# Autodesk Inventor assembly: joint4
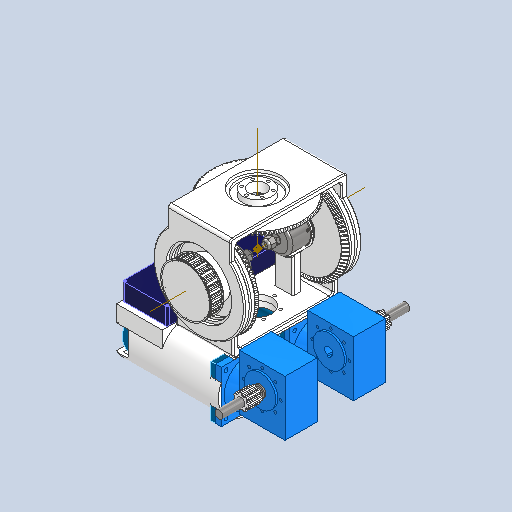
[picture p0: Inventor's stored thumbnail of the model, 512x512]
Saved by Autodesk Inventor 2025.3 (Build 293356030, 356C)
## iProperties
Created: 2025-08-31
Part Number: joint4
Document SubType Name: Assembly
Designer: MSI
Mass: 16772.4 g
Surface Area: 9850.81 cm^2
Volume: 6074.34 cm^3
Density: 2.76119 g/cm^3
Author: MSI
## Documents named in this file (14)
- C:\Users\MSI\Desktop\Project\11. 로봇팔\Robot Arm Model\Robot_Arm_6_v1\joint4.iam
- C:\Users\MSI\Desktop\Project\11. 로봇팔\Robot Arm Model\Robot_Arm_6_v1\motor_holder_1.ipt
- C:\Users\MSI\Desktop\Project\11. 로봇팔\Robot Arm Model\Robot_Arm_6_v1\NMRV30_motor.iam
- C:\Users\MSI\Desktop\Project\11. 로봇팔\Robot Arm Model\Robot_Arm_6_v1\base.ipt
- C:\Users\MSI\Desktop\Project\11. 로봇팔\Robot Arm Model\Robot_Arm_6_v1\frame.ipt
- C:\Users\MSI\Desktop\Project\11. 로봇팔\Robot Arm Model\Robot_Arm_6_v1\miter_gear_center.ipt
- C:\Users\MSI\Desktop\Project\11. 로봇팔\Robot Arm Model\Robot_Arm_6_v1\miter_gear_left.ipt
- C:\Users\MSI\Desktop\Project\11. 로봇팔\Robot Arm Model\Robot_Arm_6_v1\miter_gear_right.ipt
- C:\Users\MSI\Desktop\Project\11. 로봇팔\Robot Arm Model\Robot_Arm_6_v1\encoder.ipt
- C:\Users\MSI\Desktop\Project\11. 로봇팔\Robot Arm Model\Robot_Arm_6_v1\belt_pulley_1.ipt
- C:\Users\MSI\Desktop\Project\11. 로봇팔\Robot Arm Model\Robot_Arm_6_v1\belt_pulley_2.ipt
- C:\Users\MSI\Desktop\Project\11. 로봇팔\Robot Arm Model\Robot_Arm_6_v1\motor_shaft.ipt
- C:\Users\MSI\Desktop\Project\11. 로봇팔\Robot Arm Model\Robot_Arm_6_v1\motor_driver.ipt
- C:\Users\MSI\Desktop\Project\11. 로봇팔\Robot Arm Model\Robot_Arm_6_v1\encoder_frame.ipt
## Components (20 placed, 12 different names)
1. base:1 — 회전:1, 회전:2, 회전:3, 강체:5, 강체:15, 강체:17
2. frame:1 — 회전:1, 회전:4, 강체:6, 강체:8
3. 베벨 기어2:1 — 회전:4
4. 베벨 기어1:1 — 회전:2
5. 베벨 기어1:2 — 회전:3
6. encoder:1 — 강체:16
7. encoder:2 — 강체:14
8. NMRV30_motor:1 [sub-assembly] — 강체:3, 강체:9, 강체:11
9. NMRV30_motor:2 [sub-assembly] — 강체:4, 강체:7, 강체:10
10. motor_holder_1:1 — 강체:3, 강체:4, 강체:5, 강체:12, 강체:13
11. 동기식 풀리1:1 — 강체:7
12. 동기식 풀리2:1 — 강체:6
13. 동기식 풀리1:2 — 강체:9
14. 동기식 풀리2:2 — 강체:8
15. motor_shaft:1 — 강체:11
16. motor_shaft:2 — 강체:10
17. motor_driver:1 — 강체:13
18. motor_driver:2 — 강체:12
19. encoder_frame:1 — 강체:14, 강체:15
20. encoder_frame:2 — 강체:16, 강체:17
## Relationships (19: WeldJoint 15, RevoluteJoint 4)
- 회전:1 [RevoluteJoint]: base:1 ↔ frame:1
- 회전:2 [RevoluteJoint]: base:1 ↔ 베벨 기어1:1
- 회전:3 [RevoluteJoint]: base:1 ↔ 베벨 기어1:2
- 회전:4 [RevoluteJoint]: frame:1 ↔ 베벨 기어2:1
- 강체:16 [WeldJoint]: encoder:1 ↔ encoder_frame:2
- 강체:14 [WeldJoint]: encoder:2 ↔ encoder_frame:1
- 강체:3 [WeldJoint]: NMRV30_motor:1 ↔ motor_holder_1:1
- 강체:4 [WeldJoint]: NMRV30_motor:2 ↔ motor_holder_1:1
- 강체:5 [WeldJoint]: base:1 ↔ motor_holder_1:1
- 강체:6 [WeldJoint]: frame:1 ↔ 동기식 풀리2:1
- 강체:7 [WeldJoint] (9 mm): NMRV30_motor:2 ↔ 동기식 풀리1:1
- 강체:8 [WeldJoint]: frame:1 ↔ 동기식 풀리2:2
- 강체:9 [WeldJoint] (9 mm): NMRV30_motor:1 ↔ 동기식 풀리1:2
- 강체:10 [WeldJoint]: NMRV30_motor:2 ↔ motor_shaft:2
- 강체:11 [WeldJoint]: NMRV30_motor:1 ↔ motor_shaft:1
- 강체:12 [WeldJoint]: motor_holder_1:1 ↔ motor_driver:2
- 강체:13 [WeldJoint]: motor_holder_1:1 ↔ motor_driver:1
- 강체:15 [WeldJoint]: base:1 ↔ encoder_frame:1
- 강체:17 [WeldJoint]: base:1 ↔ encoder_frame:2
